# Autodesk Inventor assembly: 针头
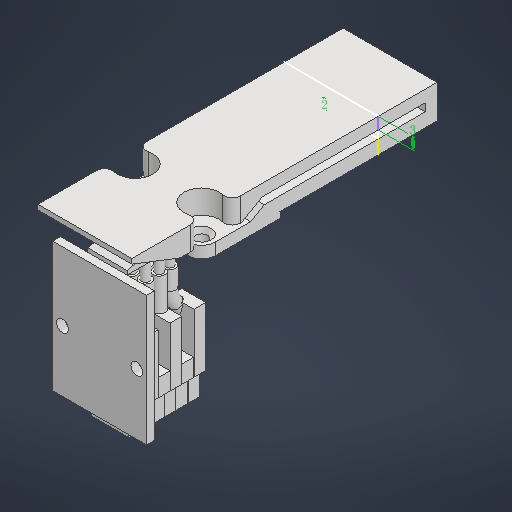
[picture p0: Inventor's stored thumbnail of the model, 512x512]
Saved by Autodesk Inventor 2025 (Build 290162000, 162)
## iProperties
Created: 2026-04-16
Part Number: 针头
Document SubType Name: Assembly
Designer: XH
Author: XH
## Documents named in this file (8)
- C:\1A_Engineering_files\braille-printer-v2\3D文件\新配件\针头.iam
- C:\1A_Engineering_files\braille-printer-v2\3D文件\新配件\针头盖.ipt
- C:\1A_Engineering_files\braille-printer-v2\3D文件\新配件\针头固定件.ipt
- C:\1A_Engineering_files\braille-printer-v2\3D文件\新配件\触点外壳.ipt
- C:\1A_Engineering_files\braille-printer-v2\3D文件\新配件\轴系按钮1.ipt
- C:\1A_Engineering_files\braille-printer-v2\3D文件\新配件\轴系按钮.ipt
- C:\1A_Engineering_files\braille-printer-v2\3D文件\新配件\轴系按钮2.ipt
- C:\1A_Engineering_files\braille-printer-v2\3D文件\新配件\轴系按钮3.ipt
## Components (9 placed, 7 different names)
1. 针头盖:1 — 配合:2, 配合:13, 配合:18, 配合:19
2. 针头固定件:1 — 配合:2, 配合:13, 配合:14, 配合:15, 配合:16
3. 触点外壳:1 — 配合:14, 配合:15, 配合:16
4. 轴系按钮1:1 — 配合:18, 配合:19, 配合:20, 表面齐平:2, 配合:21, 表面齐平:3, 表面齐平:11
5. 轴系按钮:1 — 配合:20, 表面齐平:2, 配合:22, 表面齐平:11
6. 轴系按钮2:1 — 配合:21, 配合:22, 表面齐平:3, 配合:23, 表面齐平:5, 表面齐平:8
7. 轴系按钮3:1 — 配合:23, 表面齐平:5, 配合:24, 表面齐平:6, 表面齐平:7
8. 轴系按钮3:2 — 配合:24, 表面齐平:6, 表面齐平:7, 表面齐平:8, 表面齐平:9, 表面齐平:10
9. 轴系按钮2:2 — 表面齐平:9, 表面齐平:10
## Relationships (21: Mate 12, Flush 9)
- 配合:2 [Mate]: 针头盖:1 ↔ 针头固定件:1
- 配合:13 [Mate]: 针头盖:1 ↔ 针头固定件:1
- 配合:14 [Mate]: 针头固定件:1 ↔ 触点外壳:1
- 配合:15 [Mate]: 针头固定件:1 ↔ 触点外壳:1
- 配合:16 [Mate]: 针头固定件:1 ↔ 触点外壳:1
- 配合:18 [Mate]: 针头盖:1 ↔ 轴系按钮1:1
- 配合:19 [Mate]: 针头盖:1 ↔ 轴系按钮1:1
- 配合:20 [Mate]: 轴系按钮1:1 ↔ 轴系按钮:1
- 表面齐平:2 [Flush]: 轴系按钮1:1 ↔ 轴系按钮:1
- 配合:21 [Mate]: 轴系按钮1:1 ↔ 轴系按钮2:1
- 配合:22 [Mate]: 轴系按钮:1 ↔ 轴系按钮2:1
- 表面齐平:3 [Flush]: 轴系按钮1:1 ↔ 轴系按钮2:1
- 配合:23 [Mate]: 轴系按钮2:1 ↔ 轴系按钮3:1
- 表面齐平:5 [Flush]: 轴系按钮2:1 ↔ 轴系按钮3:1
- 配合:24 [Mate]: 轴系按钮3:1 ↔ 轴系按钮3:2
- 表面齐平:6 [Flush]: 轴系按钮3:1 ↔ 轴系按钮3:2
- 表面齐平:7 [Flush]: 轴系按钮3:1 ↔ 轴系按钮3:2
- 表面齐平:8 [Flush]: 轴系按钮2:1 ↔ 轴系按钮3:2
- 表面齐平:9 [Flush]: 轴系按钮3:2 ↔ 轴系按钮2:2
- 表面齐平:10 [Flush]: 轴系按钮3:2 ↔ 轴系按钮2:2
- 表面齐平:11 [Flush]: 轴系按钮1:1 ↔ 轴系按钮:1
